# Autodesk Inventor assembly: GP4-100
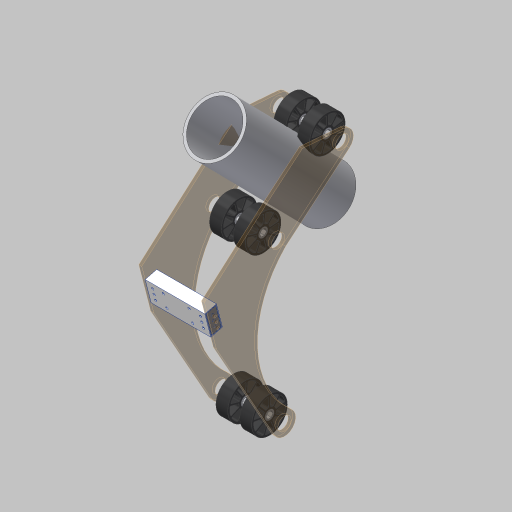
[picture p0: Inventor's stored thumbnail of the model, 512x512]
Saved by Autodesk Inventor 2023.5 (Build 275446000, 446)
## iProperties
Created: 2025-01-28
Part Number: GP4-100
Document SubType Name: Assembly
Designer: slick
Author: slick
## Documents named in this file (7)
- C:\Users\slick\OneDrive\Desktop\2025-ReefScape---CAD\Gripper\GP4\GP4-100.iam
- C:\Users\slick\OneDrive\Desktop\2025-ReefScape---CAD\Gripper\GP4\GP4-001.ipt
- C:\Users\slick\OneDrive\Desktop\2025-ReefScape---CAD\Gripper\GP4\GP4-002.ipt
- C:\Users\slick\OneDrive\Desktop\2025-ReefScape---CAD\Gripper\GP4\GP4-003.ipt
- C:\Users\slick\OneDrive\Desktop\2025-ReefScape---CAD\Gripper\GP4\GP4-003_MIR.ipt
- C:\Users\slick\OneDrive\Desktop\2025-ReefScape---CAD\Field Items\Game Pieces\GE-25500.ipt
- C:\Users\slick\OneDrive\Desktop\2025-ReefScape---CAD\COMMON PARTS\WHEELS\am-3945 3IN 500Hex Compliant Wheel REV 3.ipt
## Components (12 placed, 6 different names)
1. GP4-001:1 — Insert:1, Insert:2, Mate:2, Mate:4, Mate:6
2. GP4-002:1 — Flush:1, Flush:2, Flush:3, Mate:1, Flush:4, Flush:5, Angle:1
3. GP4-003:1 — Flush:1, Mate:1, Flush:4, Insert:1, Insert:2
4. GP4-003_MIR:1 — Flush:2, Flush:3, Flush:5, Insert:3, Insert:4
5. GP4-001:2 — Insert:3, Insert:4, Mate:7, Mate:10
6. GE-25500:1 — Angle:1
7. am-3945 3IN 500Hex Compliant Wheel REV 3:1 — Mate:5, Mate:9, Flush:6
8. am-3945 3IN 500Hex Compliant Wheel REV 3:2 — Mate:4, Mate:5, Mate:9, Flush:7, Flush:8
9. am-3945 3IN 500Hex Compliant Wheel REV 3:3 — Mate:7, Mate:8, Flush:8
10. am-3945 3IN 500Hex Compliant Wheel REV 3:4 — Mate:6, Mate:8
11. am-3945 3IN 500Hex Compliant Wheel REV 3:5 — Mate:3, Flush:7, Mate:10
12. am-3945 3IN 500Hex Compliant Wheel REV 3:6 — Mate:2, Mate:3, Flush:6
## Relationships (23: Mate 10, Flush 8, Insert 4, Angle 1)
- Flush:1: GP4-002:1 ↔ GP4-003:1
- Flush:2: GP4-002:1 ↔ GP4-003_MIR:1
- Flush:3: GP4-002:1 ↔ GP4-003_MIR:1
- Mate:1: GP4-002:1 ↔ GP4-003:1
- Flush:4: GP4-002:1 ↔ GP4-003:1
- Flush:5: GP4-002:1 ↔ GP4-003_MIR:1
- Insert:1: GP4-001:1 ↔ GP4-003:1
- Insert:2: GP4-001:1 ↔ GP4-003:1
- Insert:3: GP4-003_MIR:1 ↔ GP4-001:2
- Insert:4: GP4-003_MIR:1 ↔ GP4-001:2
- Angle:1 (150 deg): GP4-002:1 ↔ GE-25500:1
- Mate:2: GP4-001:1 ↔ am-3945 3IN 500Hex Compliant Wheel REV 3:6
- Mate:3: am-3945 3IN 500Hex Compliant Wheel REV 3:5 ↔ am-3945 3IN 500Hex Compliant Wheel REV 3:6
- Mate:4: GP4-001:1 ↔ am-3945 3IN 500Hex Compliant Wheel REV 3:2
- Mate:5: am-3945 3IN 500Hex Compliant Wheel REV 3:1 ↔ am-3945 3IN 500Hex Compliant Wheel REV 3:2
- Mate:6: GP4-001:1 ↔ am-3945 3IN 500Hex Compliant Wheel REV 3:4
- Mate:7: GP4-001:2 ↔ am-3945 3IN 500Hex Compliant Wheel REV 3:3
- Mate:8 (25.4 mm): am-3945 3IN 500Hex Compliant Wheel REV 3:3 ↔ am-3945 3IN 500Hex Compliant Wheel REV 3:4
- Mate:9 (25.4 mm): am-3945 3IN 500Hex Compliant Wheel REV 3:1 ↔ am-3945 3IN 500Hex Compliant Wheel REV 3:2
- Flush:6: am-3945 3IN 500Hex Compliant Wheel REV 3:1 ↔ am-3945 3IN 500Hex Compliant Wheel REV 3:6
- Flush:7: am-3945 3IN 500Hex Compliant Wheel REV 3:2 ↔ am-3945 3IN 500Hex Compliant Wheel REV 3:5
- Mate:10 (25.4 mm): GP4-001:2 ↔ am-3945 3IN 500Hex Compliant Wheel REV 3:5
- Flush:8: am-3945 3IN 500Hex Compliant Wheel REV 3:2 ↔ am-3945 3IN 500Hex Compliant Wheel REV 3:3
